# Autodesk Inventor assembly: JB_CAD_Final_Assembly
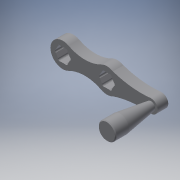
[picture p0: Inventor's stored thumbnail of the model, 180x180]
Saved by Autodesk Inventor 2016 (Build 200138000, 138)
## iProperties
Created: 2018-06-18
Part Number: JB_CAD_Final_Assembly
Document SubType Name: Assembly
Designer: Student
Author: Student
## Documents named in this file (3)
- C:\Users\Student\Documents\Derek Code and Projects\Autodesk\JB_CAD_Final_Assembly.iam
- C:\Users\Student\Documents\Derek Code and Projects\Autodesk\JB_CAD_FinalPt1.ipt
- C:\Users\Student\Documents\Derek Code and Projects\Autodesk\JB_CAD_FinalPt2.ipt
## Components (2 placed, 2 different names)
1. JB_CAD_FinalPt1:1 — Rotational:1
2. JB_CAD_FinalPt2:1 — Rotational:1
## Relationships (1: RevoluteJoint 1)
- Rotational:1 [RevoluteJoint]: JB_CAD_FinalPt1:1 ↔ JB_CAD_FinalPt2:1
